# Autodesk Inventor assembly: room
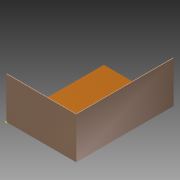
[picture p0: Inventor's stored thumbnail of the model, 180x180]
Saved by Autodesk Inventor 2015 (Build 190159000, 159)
## iProperties
Created: 2015-10-19
Part Number: room
Document SubType Name: Assembly
Designer: omae
Author: omae
## Documents named in this file (4)
- C:\Users\omae\Desktop\研究室\論文・資料\ROS\kitchen\kitchen\CAD\room.iam
- C:\Users\omae\Desktop\研究室\論文・資料\ROS\kitchen\toolinstall\homeIsland\summerSeminar\floor.ipt
- C:\Users\omae\Desktop\研究室\論文・資料\ROS\kitchen\toolinstall\homeIsland\summerSeminar\wall.ipt
- C:\Users\omae\Desktop\研究室\論文・資料\ROS\kitchen\toolinstall\homeIsland\summerSeminar\wall2.ipt
## Components (3 placed, 3 different names)
1. floor:1 — メイト:1, メイト:4, メイト:6, メイト:9
2. wall:1 — メイト:5, メイト:6, メイト:7
3. wall2:1 — メイト:2, メイト:3, メイト:4, メイト:7, メイト:8
## Relationships (9: Mate 9)
- メイト:1 [Mate]: floor:1
- メイト:2 [Mate]: wall2:1
- メイト:3 [Mate]: wall2:1
- メイト:4 [Mate]: floor:1 ↔ wall2:1
- メイト:5 [Mate]: wall:1
- メイト:6 [Mate]: floor:1 ↔ wall:1
- メイト:7 [Mate]: wall:1 ↔ wall2:1
- メイト:8 [Mate]: wall2:1
- メイト:9 [Mate]: floor:1
